# Autodesk Inventor assembly: Ensamblaje1
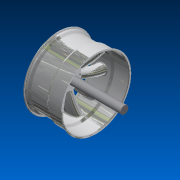
[picture p0: Inventor's stored thumbnail of the model, 180x180]
Saved by Autodesk Inventor 2013 (Build 170138000, 138)
## iProperties
Created: 2013-10-20
Part Number: Ensamblaje1
Document SubType Name: Assembly
Designer: Miguel
Author: Miguel
## Documents named in this file (3)
- E:\Mis Documentos\Inventor\llanta\Ensamblaje1.iam
- E:\Mis Documentos\Inventor\llanta\llanta.ipt
- E:\Mis Documentos\Inventor\llanta\eje.ipt
## Components (2 placed, 2 different names)
1. llanta:1 — Coincidencia:1, Nivelación:1
2. eje:1 — Coincidencia:1, Nivelación:1
## Relationships (2: Mate 1, Flush 1)
- Coincidencia:1 [Mate]: llanta:1 ↔ eje:1
- Nivelación:1 [Flush]: llanta:1 ↔ eje:1
